# Autodesk Inventor assembly: Assembly_Guinardia_V4
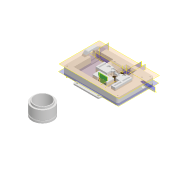
[picture p0: Inventor's stored thumbnail of the model, 180x180]
Saved by Autodesk Inventor 2022 (Build 260153000, 153)
## iProperties
Created: 2023-01-07
Part Number: Assembly_Guinardia_V4
Document SubType Name: Assembly
Designer: diederichbenedict
Author: diederichbenedict
## Documents named in this file (5)
- C:\Users\diederichbenedict\Dropbox\Dokumente\Promotion\PROJECTS\HoLiSheet\INVENTOR\Assembly_Guinardia_V4.iam
- C:\Users\diederichbenedict\Dropbox\Dokumente\Promotion\PROJECTS\HoLiSheet\INVENTOR\10_Wellplate_base_v3.ipt
- C:\Users\diederichbenedict\Dropbox\Dokumente\Promotion\PROJECTS\HoLiSheet\INVENTOR\Assemlby_Scanner_v1.iam
- C:\Users\diederichbenedict\Dropbox\Dokumente\Promotion\PROJECTS\HoLiSheet\INVENTOR\11_Wellplatespacer.ipt
- C:\Users\diederichbenedict\Dropbox\Dokumente\Promotion\PROJECTS\HoLiSheet\INVENTOR\00_microscope_turret.ipt
## Components (4 placed, 4 different names)
1. 10_Wellplate_base_v3:1 — Passend:1, Passend:2, Winkel:1, Einfügen:1, Winkel:2, Fluchtend:1, Fluchtend:2
2. Assemlby_Scanner_v1:1 [sub-assembly] — Passend:1, Passend:2, Winkel:1, Fluchtend:1, Fluchtend:2
3. 11_Wellplatespacer:1 — Einfügen:1, Winkel:2
4. 00_microscope_turret:1
## Relationships (7: Mate 2, Angle 2, Flush 2, Insert 1)
- Passend:1 [Mate]: 10_Wellplate_base_v3:1 ↔ Assemlby_Scanner_v1:1
- Passend:2 [Mate] (1.4 mm): 10_Wellplate_base_v3:1 ↔ Assemlby_Scanner_v1:1
- Winkel:1 [Angle] (0 deg): 10_Wellplate_base_v3:1 ↔ Assemlby_Scanner_v1:1
- Einfügen:1 [Insert]: 10_Wellplate_base_v3:1 ↔ 11_Wellplatespacer:1
- Winkel:2 [Angle] (180 deg): 10_Wellplate_base_v3:1 ↔ 11_Wellplatespacer:1
- Fluchtend:1 [Flush]: 10_Wellplate_base_v3:1 ↔ Assemlby_Scanner_v1:1
- Fluchtend:2 [Flush]: 10_Wellplate_base_v3:1 ↔ Assemlby_Scanner_v1:1
